# Autodesk Inventor assembly: Assembly2
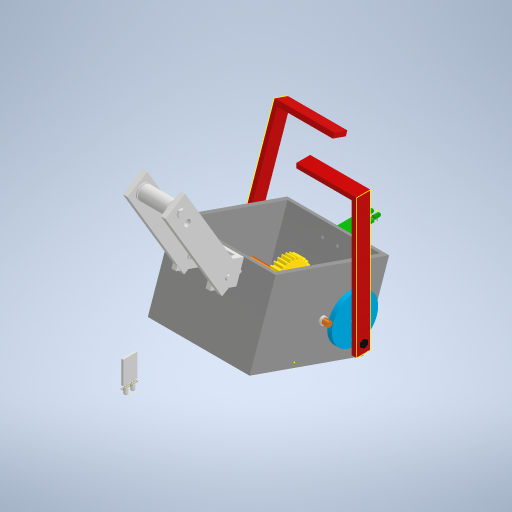
[picture p0: Inventor's stored thumbnail of the model, 512x512]
Saved by Autodesk Inventor 2023 (Build 270158000, 158)
## iProperties
Created: 2022-06-16
Part Number: Assembly2
Document SubType Name: Assembly
Designer: TRIVENI MAGADUM
Author: TRIVENI MAGADUM
## Documents named in this file (15)
- D:\Assembly2.iam
- D:\big gear.ipt
- D:\container3.ipt
- D:\DC MOTOR1.ipt
- D:\Part4.ipt
- D:\small gear.ipt
- D:\cube.ipt
- D:\Part1.ipt
- D:\Part2.ipt
- D:\Part3.ipt
- D:\Screw 5 mm.ipt
- D:\Final assembly 3.iam
- D:\Screw 3mm.ipt
- D:\Bolt 3mm.ipt
- D:\IR Sensor.ipt
## Components (35 placed, 14 different names)
1. container3:1 — Insert:1, Insert:2, Insert:3, Insert:4, Mate:1, Flush:1, Insert:14, Insert:15, Insert:21, Insert:28, Insert:31, Insert:32, Angle:1, Mate:2
2. big gear:1 — Insert:5
3. big gear:2 — Insert:1, Rotation:1, Rotation:2
4. Part4:1 — Insert:2, Rotation:1, Rotation:2, Rotation:3
5. Part4:2 — Insert:4, Rotation:3, Rotational:1, Insert:7, Insert:11
6. small gear:2 — Insert:3
7. DC MOTOR1:2 — Tangent:1, Insert:5
8. cube:1 — Mate:1, Tangent:1, Flush:1
9. Part1:1 — Rotational:1
10. Part1:4 — Insert:7
11. Part1:5 — Insert:11
12. Part1:13 — Insert:14
13. Part1:15 — Insert:17
14. Part1:16 — Insert:15, Insert:16
15. Part2:1 — Insert:16, Insert:17, Insert:18
16. Part2:2 — Insert:22, Insert:23, Insert:24
17. Part1:17 — Insert:23
18. Part1:18 — Insert:21, Insert:22
19. Part1:19 — Insert:19, Insert:20
20. Part1:20 — Insert:18, Insert:19
21. Part3:1 — Insert:20, Insert:27
22. Part1:22 — Insert:25, Rotational:2
23. Part1:23 — Insert:24, Insert:25
24. Part3:2 — Rotational:2, Insert:26, Angle:1
25. Screw 5 mm:1 — Insert:26
26. Screw 5 mm:2 — Insert:27
27. Final assembly 3:1 [sub-assembly] — Insert:28, Insert:29, Insert:30, Insert:33, Insert:34
28. Screw 3mm:1 — Insert:30
29. Screw 3mm:2 — Insert:29
30. Bolt 3mm:1 — Insert:31
31. Bolt 3mm:2 — Insert:32
32. Bolt 3mm:3 — Insert:33
33. Bolt 3mm:4 — Insert:34
34. IR Sensor:2 — Mate:2
35. IR Sensor:3
## Relationships (38: Insert 28, RelateRotation 3, Mate 2, RevoluteJoint 2, Tangent 1, Flush 1, Angle 1)
- Insert:1 (57 mm): container3:1 ↔ big gear:2
- Insert:2 (-10 mm): container3:1 ↔ Part4:1
- Insert:3 (57 mm): container3:1 ↔ small gear:2
- Insert:4 (-10 mm): container3:1 ↔ Part4:2
- Rotation:1 [RelateRotation] (20 ul): big gear:2 ↔ Part4:1
- Rotation:2 [RelateRotation] (1 ul): big gear:2 ↔ Part4:1
- Mate:1: container3:1 ↔ cube:1
- Tangent:1: DC MOTOR1:2 ↔ cube:1
- Insert:5 (-10 mm): big gear:1 ↔ DC MOTOR1:2
- Flush:1: container3:1 ↔ cube:1
- Rotation:3 [RelateRotation] (1 ul): Part4:1 ↔ Part4:2
- Rotational:1 [RevoluteJoint] (-11 mm): Part4:2 ↔ Part1:1
- Insert:7 (-13 mm): Part4:2 ↔ Part1:4
- Insert:11 (-11 mm): Part4:2 ↔ Part1:5
- Insert:14: container3:1 ↔ Part1:13
- Insert:15: container3:1 ↔ Part1:16
- Insert:16: Part1:16 ↔ Part2:1
- Insert:17: Part1:15 ↔ Part2:1
- Insert:18: Part2:1 ↔ Part1:20
- Insert:19: Part1:19 ↔ Part1:20
- Insert:20: Part1:19 ↔ Part3:1
- Insert:21: container3:1 ↔ Part1:18
- Insert:22: Part2:2 ↔ Part1:18
- Insert:23: Part2:2 ↔ Part1:17
- Insert:24: Part2:2 ↔ Part1:23
- Insert:25: Part1:22 ↔ Part1:23
- Rotational:2 [RevoluteJoint]: Part1:22 ↔ Part3:2
- Insert:26 (-15 mm): Part3:2 ↔ Screw 5 mm:1
- Insert:27 (-15 mm): Part3:1 ↔ Screw 5 mm:2
- Insert:28: container3:1 ↔ Final assembly 3:1
- Insert:29 (-14.5 mm): Final assembly 3:1 ↔ Screw 3mm:2
- Insert:30 (-14.5 mm): Final assembly 3:1 ↔ Screw 3mm:1
- Insert:31: container3:1 ↔ Bolt 3mm:1
- Insert:32: container3:1 ↔ Bolt 3mm:2
- Insert:33: Final assembly 3:1 ↔ Bolt 3mm:3
- Insert:34: Final assembly 3:1 ↔ Bolt 3mm:4
- Angle:1 (0 deg): container3:1 ↔ Part3:2
- Mate:2: container3:1 ↔ IR Sensor:2
